# Autodesk Inventor assembly: 61814
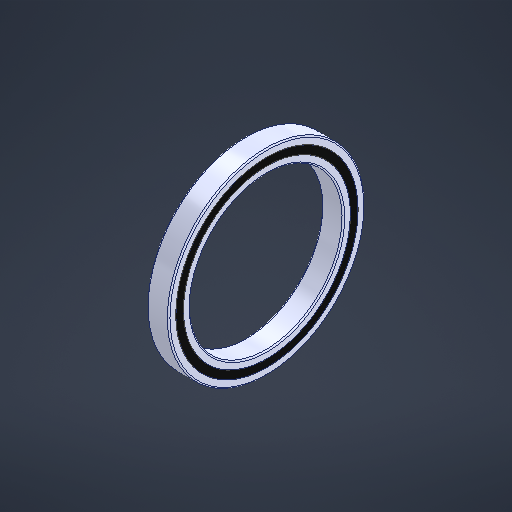
[picture p0: Inventor's stored thumbnail of the model, 512x512]
Saved by Autodesk Inventor 2025.2 (Build 292293000, 293)
## iProperties
Created: 2025-07-08
Part Number: 61814
Document SubType Name: Assembly
Designer: Tiago
Sending System: SolidWorks 2015
Last Author: tpomodeler
Last Saved: 2025-07-08
CG: Sheet metal
NO_OF_ROWS: 1
SUPPLIER: SKF
SLNG_TYPE: -
BORE_D: 70
DYN_LOAD_C: 12.4
MAT_BEAR: Bearing steel
RD_INT_CLR: CN
COAT: Without
OUTSIDE_D: 90
DESIGN: Deep groove ball bearings
WIDTH_B: 10
SLNG: Without
FL_SLTS: Without
REFERENCE: 61814
SKF_CLASS: -
LIM_SPEED: 9000
DESCR: Deep groove ball bearing
TraceParts.PartTitle: Deep groove ball bearings
TRACEPARTS: TRACEPARTS
TraceParts.PartLanguage: en
TraceParts.InstanceId: 34-21082024-09662556PT1MBL83HT9XA8PPZJLIIU2
TraceParts.PartNumber: 34-21082024-096625
TraceParts.PartVersion: 1.2.1
TYPE: CATPART
Title: Deep groove ball bearings
Author: TraceParts
## Documents named in this file (6)
- C:\Users\Tiago\Documents\Inventor\Exp. Braço v1\Rolamento TestBR\61814\61814\61814.iam
- C:\Users\Tiago\Documents\Inventor\Exp. Braço v1\Rolamento TestBR\61814\61814\61814_01.ipt
- C:\Users\Tiago\Documents\Inventor\Exp. Braço v1\Rolamento TestBR\61814\61814\61814_02.ipt
- C:\Users\Tiago\Documents\Inventor\Exp. Braço v1\Rolamento TestBR\61814\61814\61814_03.ipt
- C:\Users\Tiago\Documents\Inventor\Exp. Braço v1\Rolamento TestBR\Part7.ipt
- Rubber_61814.ipt
## Components (5 placed, 4 different names)
1. 61814_01:1 — Mate:1, Flush:1, Flush:4, Flush:5
2. 61814_02:1 — Mate:1, Mate:2, Flush:1, Mate:3, Mate:4
3. 61814_03:1 — Mate:2, Flush:2
4. Rubber_61814:1 — Mate:3, Flush:4
5. Rubber_61814:2 — Mate:4, Flush:5
## Relationships (8: Mate 4, Flush 4)
- Mate:1: 61814_01:1 ↔ 61814_02:1
- Mate:2: 61814_02:1 ↔ 61814_03:1
- Flush:1: 61814_01:1 ↔ 61814_02:1
- Flush:2: 61814_03:1
- Mate:3: 61814_02:1 ↔ Rubber_61814:1
- Flush:4: 61814_01:1 ↔ Rubber_61814:1
- Mate:4: 61814_02:1 ↔ Rubber_61814:2
- Flush:5: 61814_01:1 ↔ Rubber_61814:2
